# Autodesk Inventor assembly: Wrist
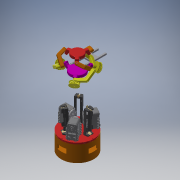
[picture p0: Inventor's stored thumbnail of the model, 180x180]
Saved by Autodesk Inventor 2019 (Build 230136000, 136)
## iProperties
Created: 2022-08-01
Part Number: Wrist
Document SubType Name: Assembly
Designer: zreik
Author: zreik
## Documents named in this file (4)
- D:\Documents\HIAST\4th year\4th Year Project\Design\Wrist.iam
- D:\Documents\HIAST\4th year\4th Year Project\Design\BottomPart.iam
- D:\Documents\HIAST\4th year\4th Year Project\Design\SPM.iam
- D:\Documents\HIAST\4th year\4th Year Project\Design\Bridge.ipt
## Components (3 placed, 3 different names)
1. BottomPart:1 [sub-assembly] — Flush:1, Flush:2, Flush:3, Mate:1
2. SPM:1 [sub-assembly] — Mate:1
3. Bridge:1
## Relationships (4: Flush 3, Mate 1)
- Flush:1: BottomPart:1
- Flush:2: BottomPart:1
- Flush:3: BottomPart:1
- Mate:1: BottomPart:1 ↔ SPM:1
